# Autodesk Inventor assembly: Head
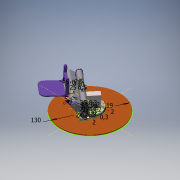
[picture p0: Inventor's stored thumbnail of the model, 180x180]
Saved by Autodesk Inventor 2018.3 (Build 223284000, 284)
## iProperties
Created: 2018-05-16
Part Number: Head
Material: Generisch
Document SubType Name: Assembly
Designer: JochenAlt
Author: JochenAlt
## Documents named in this file (11)
- D:\Projects\Donna\CAD\Head.iam
- D:\Projects\Donna\CAD\Stewart-Head.ipt
- D:\Projects\Donna\CAD\Mouth-Base.ipt
- D:\Projects\Donna\CAD\Servo-KST-DS215MG.ipt
- D:\Projects\Donna\CAD\Rillenkugellager 61707-2RS1.iam
- D:\Projects\Donna\CAD\Mouth-Height-Lever-front.ipt
- D:\Projects\Donna\CAD\Ball-Joint-male.ipt
- D:\Projects\Donna\CAD\Servo-Arm-Lip.ipt
- D:\Projects\Donna\CAD\Servo-Arm-Mouth.ipt
- C:\Users\JochenAlt\Documents\Inventor\Content Center Files\R2018\de-DE\BS 290 SKF(30)\BS 290 SKF - SKF 623.ipt
- D:\Projects\Donna\CAD\Mouth-Turn-Disk.ipt
## Components (18 placed, 9 different names)
1. Stewart-Plate-Head:1 — Passend:1, Passend:2, Passend:3, Passend:6, Passend:7, Passend:18, Passend:19, Passend:20, Passend:21, Passend:22, Passend:23, Passend:24, Passend:25, Passend:26, Passend:27, Passend:28, Passend:29
2. Mouth-Base:1 — Passend:1, Passend:2, Passend:4, Passend:8, Passend:30, Passend:31, Passend:32, Passend:33, Passend:34, Passend:35
3. Servo-KST-DS215MG:1 — Passend:3, Passend:4, Passend:8, Passend:49, Passend:50
4. Rillenkugellager 61707-2RS1:1 [sub-assembly] — Passend:6, Passend:7
5. Mouth-Height-Lever:2 — Passend:46, Passend:47
6. ball joint:1 — Passend:18, Passend:29
7. ball joint:2 — Passend:19, Passend:28
8. ball joint:3 — Passend:23, Passend:25
9. ball joint:4 — Passend:22, Passend:24
10. ball joint:5 — Passend:21, Passend:27
11. ball joint:6 — Passend:20, Passend:26
12. Servo-KST-DS215MG:2 — Passend:33, Passend:34, Passend:35, Passend:38, Passend:39
13. Servo-KST-DS215MG:3 — Passend:30, Passend:31, Passend:32, Passend:36, Passend:37
14. ServoArm:1 — Passend:36, Passend:37, Passend:40, Passend:41, Passend:46, Passend:47
15. ServoArm:2 — Passend:38, Passend:39, Passend:44, Passend:45
16. BS 290 SKF 623:1 — Passend:40, Passend:41
17. BS 290 SKF 623:2 — Passend:44, Passend:45
18. Mouth-Turn-Disk:1 — Passend:49, Passend:50
## Relationships (37: Mate 37)
- Passend:1 [Mate]: Stewart-Plate-Head:1 ↔ Mouth-Base:1
- Passend:2 [Mate] (5 mm): Stewart-Plate-Head:1 ↔ Mouth-Base:1
- Passend:3 [Mate]: Stewart-Plate-Head:1 ↔ Servo-KST-DS215MG:1
- Passend:4 [Mate]: Mouth-Base:1 ↔ Servo-KST-DS215MG:1
- Passend:6 [Mate]: Stewart-Plate-Head:1 ↔ Rillenkugellager 61707-2RS1:1
- Passend:7 [Mate]: Stewart-Plate-Head:1 ↔ Rillenkugellager 61707-2RS1:1
- Passend:8 [Mate]: Mouth-Base:1 ↔ Servo-KST-DS215MG:1
- Passend:18 [Mate]: Stewart-Plate-Head:1 ↔ ball joint:1
- Passend:19 [Mate]: Stewart-Plate-Head:1 ↔ ball joint:2
- Passend:20 [Mate]: Stewart-Plate-Head:1 ↔ ball joint:6
- Passend:21 [Mate]: Stewart-Plate-Head:1 ↔ ball joint:5
- Passend:22 [Mate]: Stewart-Plate-Head:1 ↔ ball joint:4
- Passend:23 [Mate]: Stewart-Plate-Head:1 ↔ ball joint:3
- Passend:24 [Mate]: Stewart-Plate-Head:1 ↔ ball joint:4
- Passend:25 [Mate]: Stewart-Plate-Head:1 ↔ ball joint:3
- Passend:26 [Mate]: Stewart-Plate-Head:1 ↔ ball joint:6
- Passend:27 [Mate]: Stewart-Plate-Head:1 ↔ ball joint:5
- Passend:28 [Mate]: Stewart-Plate-Head:1 ↔ ball joint:2
- Passend:29 [Mate]: Stewart-Plate-Head:1 ↔ ball joint:1
- Passend:30 [Mate]: Mouth-Base:1 ↔ Servo-KST-DS215MG:3
- Passend:31 [Mate]: Mouth-Base:1 ↔ Servo-KST-DS215MG:3
- Passend:32 [Mate]: Mouth-Base:1 ↔ Servo-KST-DS215MG:3
- Passend:33 [Mate]: Mouth-Base:1 ↔ Servo-KST-DS215MG:2
- Passend:34 [Mate]: Mouth-Base:1 ↔ Servo-KST-DS215MG:2
- Passend:35 [Mate]: Mouth-Base:1 ↔ Servo-KST-DS215MG:2
- Passend:36 [Mate]: Servo-KST-DS215MG:3 ↔ ServoArm:1
- Passend:37 [Mate] (2.6 mm): Servo-KST-DS215MG:3 ↔ ServoArm:1
- Passend:38 [Mate]: Servo-KST-DS215MG:2 ↔ ServoArm:2
- Passend:39 [Mate] (2.6 mm): Servo-KST-DS215MG:2 ↔ ServoArm:2
- Passend:40 [Mate]: ServoArm:1 ↔ BS 290 SKF 623:1
- Passend:41 [Mate]: ServoArm:1 ↔ BS 290 SKF 623:1
- Passend:44 [Mate]: ServoArm:2 ↔ BS 290 SKF 623:2
- Passend:45 [Mate]: ServoArm:2 ↔ BS 290 SKF 623:2
- Passend:46 [Mate]: Mouth-Height-Lever:2 ↔ ServoArm:1
- Passend:47 [Mate] (0.5 mm): Mouth-Height-Lever:2 ↔ ServoArm:1
- Passend:49 [Mate] (2.6 mm): Servo-KST-DS215MG:1 ↔ Mouth-Turn-Disk:1
- Passend:50 [Mate]: Servo-KST-DS215MG:1 ↔ Mouth-Turn-Disk:1
